# Autodesk Inventor assembly: MotorPhotogateAssembly
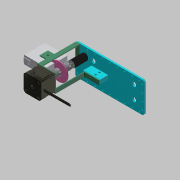
[picture p0: Inventor's stored thumbnail of the model, 180x180]
Saved by Autodesk Inventor 2018 (Build 220112000, 112)
## iProperties
Created: 2019-07-16
Part Number: MotorPhotogateAssembly
Document SubType Name: Assembly
Designer: mkivekas
Author: mkivekas
## Documents named in this file (8)
- \\cern.ch\dfs\Users\m\mkivekas\Documents\Inventor\MotorPhotogateAssembly.iam
- \\cern.ch\dfs\Users\m\mkivekas\Documents\Inventor\MotorSupport.ipt
- \\cern.ch\dfs\Users\m\mkivekas\Documents\Inventor\PhotogateCover.ipt
- \\cern.ch\dfs\Users\m\mkivekas\Documents\Inventor\PAC-SLI\Furnace drive block\PAC-SLI furnace Rv6 base.ipt
- \\cern.ch\dfs\Users\m\mkivekas\Documents\Inventor\QSH4218-35rev2.ipt
- \\cern.ch\dfs\Users\m\mkivekas\Documents\Inventor\133601.ipt
- \\cern.ch\dfs\Users\m\mkivekas\Documents\Inventor\725.16.ipt
- \\cern.ch\dfs\Users\m\mkivekas\Documents\Inventor\EncoderDisk.ipt
## Components (8 placed, 7 different names)
1. MotorSupport:1 — Mate:3, Mate:4, Mate:5, Mate:11
2. PhotogateCover:1 — Mate:17
3. PAC-SLI furnace Rv6 base:1 — Mate:11, Mate:12
4. QSH4218-35rev2:1 — Mate:3, Mate:4, Mate:5, Mate:13
5. 133601:1 — Mate:12
6. 725.16:1 — Mate:15
7. 725.16:2 — Mate:16
8. EncoderDisk:1 — Mate:13, Mate:15, Mate:16, Mate:17
## Relationships (9: Mate 9)
- Mate:3: MotorSupport:1 ↔ QSH4218-35rev2:1
- Mate:4: MotorSupport:1 ↔ QSH4218-35rev2:1
- Mate:5: MotorSupport:1 ↔ QSH4218-35rev2:1
- Mate:11: MotorSupport:1 ↔ PAC-SLI furnace Rv6 base:1
- Mate:12: PAC-SLI furnace Rv6 base:1 ↔ 133601:1
- Mate:13: QSH4218-35rev2:1 ↔ EncoderDisk:1
- Mate:15: 725.16:1 ↔ EncoderDisk:1
- Mate:16: 725.16:2 ↔ EncoderDisk:1
- Mate:17: PhotogateCover:1 ↔ EncoderDisk:1
